# Autodesk Inventor assembly: SkateScooter2
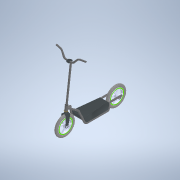
[picture p0: Inventor's stored thumbnail of the model, 180x180]
Saved by Autodesk Inventor 2022 (Build 260153000, 153)
## iProperties
Created: 2023-10-17
Part Number: SkateScooter2
Document SubType Name: Assembly
Designer: yadav
Author: yadav
## Documents named in this file (10)
- C:\Users\yadav\Documents\Inventor\SkateScooter2\SkateScooter2.iam
- C:\Users\yadav\Documents\Inventor\SkateScooter2\Fork.ipt
- C:\Users\yadav\Documents\Inventor\SkateScooter2\cubierta.ipt
- C:\Users\yadav\Documents\Inventor\SkateScooter2\Ensamblaje llanta_Predeterminado.iam
- C:\Users\yadav\Documents\Inventor\SkateScooter2\Main Frame.ipt
- C:\Users\yadav\Documents\Inventor\SkateScooter2\Handle Bar.ipt
- C:\Users\yadav\Documents\Inventor\SkateScooter2\Battery Box.ipt
- C:\Users\yadav\Documents\Inventor\SkateScooter2\Battery Box Lid.ipt
- C:\Users\yadav\Documents\Inventor\SkateScooter2\Handle.ipt
- C:\Users\yadav\Documents\Inventor\SkateScooter2\pipa manubrio 22mm diam_Predeterminado.ipt
## Components (11 placed, 9 different names)
1. Fork:1 — Flush:1, Flush:3, Mate:2, Flush:4, Flush:5
2. Main Frame:1 — Flush:3, Mate:2, Flush:4
3. Handle Bar:1 — Flush:5, Mate:3
4. Battery Box:1
5. Battery Box Lid:1
6. Handle:1 — Mate:4
7. pipa manubrio 22mm diam_Predeterminado:1 — Mate:3, Mate:4
8. Ensamblaje llanta_Predeterminado:1 [sub-assembly] — Mate:1
9. cubierta:2 — Mate:1
10. Ensamblaje llanta_Predeterminado:2 [sub-assembly]
11. cubierta:3
## Component patterns: (2 elements, first: Ensamblaje llanta_Predeterminado:1 + cubierta:2)
## Relationships (8: Flush 4, Mate 4)
- Flush:1: Fork:1
- Mate:1: Ensamblaje llanta_Predeterminado:1 ↔ cubierta:2
- Flush:3 (10 mm): Fork:1 ↔ Main Frame:1
- Mate:2: Fork:1 ↔ Main Frame:1
- Flush:4: Fork:1 ↔ Main Frame:1
- Flush:5 (10 mm): Fork:1 ↔ Handle Bar:1
- Mate:3: Handle Bar:1 ↔ pipa manubrio 22mm diam_Predeterminado:1
- Mate:4: Handle:1 ↔ pipa manubrio 22mm diam_Predeterminado:1
